# Autodesk Inventor assembly: ASM IMU
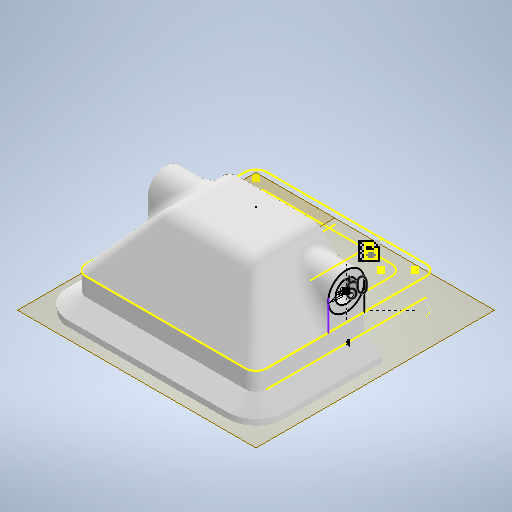
[picture p0: Inventor's stored thumbnail of the model, 512x512]
Saved by Autodesk Inventor 2025.2 (Build 292293000, 293)
## iProperties
Created: 2024-11-14
Part Number: ASM IMU
Document SubType Name: Assembly
Designer: matss
Author: matss
## Documents named in this file (5)
- C:\Users\matss\Documents\.Studium\Health Device\CAD\Wearable-Health-Device\ASM IMU.iam
- C:\Users\matss\Documents\.Studium\Health Device\CAD\Wearable-Health-Device\MPU6050 v2\MPU6050 v2\MPU6050 v2.ipt
- C:\Users\matss\Documents\.Studium\Health Device\CAD\Wearable-Health-Device\IMU_Base_T-Shirt.ipt
- C:\Users\matss\Documents\.Studium\Health Device\CAD\Wearable-Health-Device\IMU_mount_baseplate.ipt
- C:\Users\matss\Documents\.Studium\Health Device\CAD\Wearable-Health-Device\IMU_mount_cover.ipt
## Components (4 placed, 4 different names)
1. MPU6050 v2:1 — Mate:8, Angle:2, Mate:9
2. IMU_Base_T-Shirt:1 — Mate:1, Mate:2, Mate:3, Mate:4, Angle:1, Mate:5, Mate:6, Mate:7, Mate:11
3. IMU_mount_baseplate:1 — Mate:5, Mate:6, Mate:7, Mate:8, Mate:9
4. IMU_mount_cover:1 — Mate:10, Mate:11, Mate:12
## Relationships (14: Mate 12, Angle 2)
- Mate:1: IMU_Base_T-Shirt:1
- Mate:2: IMU_Base_T-Shirt:1
- Mate:3: IMU_Base_T-Shirt:1
- Mate:4: IMU_Base_T-Shirt:1
- Angle:1 (0 deg): IMU_Base_T-Shirt:1
- Mate:5: IMU_Base_T-Shirt:1 ↔ IMU_mount_baseplate:1
- Mate:6: IMU_Base_T-Shirt:1 ↔ IMU_mount_baseplate:1
- Mate:7: IMU_Base_T-Shirt:1 ↔ IMU_mount_baseplate:1
- Mate:8: MPU6050 v2:1 ↔ IMU_mount_baseplate:1
- Angle:2 (90 deg): MPU6050 v2:1
- Mate:9 (2 mm): MPU6050 v2:1 ↔ IMU_mount_baseplate:1
- Mate:10: IMU_mount_cover:1
- Mate:11: IMU_Base_T-Shirt:1 ↔ IMU_mount_cover:1
- Mate:12: IMU_mount_cover:1
